# Autodesk Inventor assembly: Banda
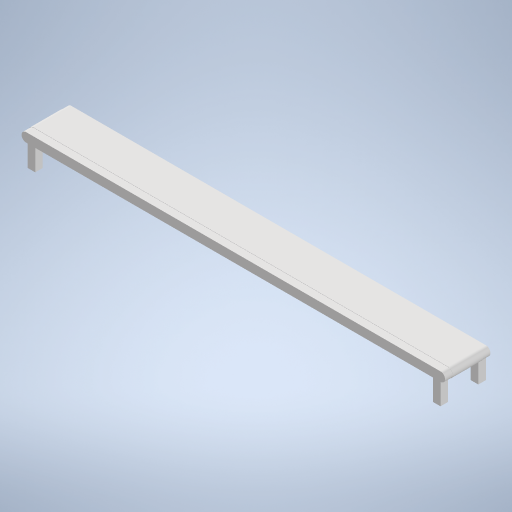
[picture p0: Inventor's stored thumbnail of the model, 512x512]
Saved by Autodesk Inventor 2024 (Build 280153000, 153)
## iProperties
Created: 2024-06-28
Part Number: Banda
Document SubType Name: Assembly
Designer: USER
Author: USER
## Documents named in this file (3)
- C:\Users\USER\Documents\APM\CAD\BandasNX\Banda.iam
- C:\Users\USER\Documents\APM\CAD\BandasNX\BandaLona.ipt
- C:\Users\USER\Documents\APM\CAD\BandasNX\SoporteBanda.ipt
## Components (2 placed, 2 different names)
1. BandaLona:1 — Coincidencia:2, Coincidencia:3
2. SoporteBanda:1 — Coincidencia:2, Coincidencia:3
## Relationships (2: Mate 2)
- Coincidencia:2 [Mate]: BandaLona:1 ↔ SoporteBanda:1
- Coincidencia:3 [Mate]: BandaLona:1 ↔ SoporteBanda:1
